# Autodesk Inventor assembly: Final Full Assembly
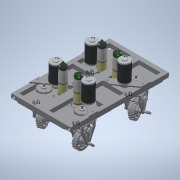
[picture p0: Inventor's stored thumbnail of the model, 180x180]
Saved by Autodesk Inventor 2021 (Build 250183000, 183)
## iProperties
Created: 2018-07-11
Part Number: Final Full Assembly
Document SubType Name: Assembly
Designer: Mortem
Author: Mortem
## Documents named in this file (19)
- C:\Users\PC\Documents\161_VS300_CAD\Final Full Assembly.iam
- F:\GrabCAD\Personal\3D Printed Swerve JP FIRST ATTEMPT\Swerve v4\Test Frame V4.iam
- F:\GrabCAD\Personal\3D Printed Swerve JP FIRST ATTEMPT\Swerve v4\Bottom Plate.ipt
- F:\GrabCAD\Personal\3D Printed Swerve JP FIRST ATTEMPT\Swerve v4\Module Seperate.iam
- F:\GrabCAD\Personal\3D Printed Swerve JP FIRST ATTEMPT\Swerve v4\56t.ipt
- F:\GrabCAD\Personal\3D Printed Swerve JP FIRST ATTEMPT\Swerve v4\cim power spacer.ipt
- F:\GrabCAD\Personal\3D Printed Swerve JP FIRST ATTEMPT\Swerve v4\am-2300+Collar+Clamp,+0.375''+Hex+Bore,+Aluminum.iam
- F:\GrabCAD\Personal\3D Printed Swerve JP FIRST ATTEMPT\Swerve v4\PG71 turning motor.iam
- F:\GrabCAD\Personal\3D Printed Swerve JP FIRST ATTEMPT\Swerve v4\New turning gear.ipt
- F:\GrabCAD\Personal\3D Printed Swerve JP FIRST ATTEMPT\Swerve v4\am-0255+2.5inch+CIM+Motor.ipt
- F:\GrabCAD\Personal\3D Printed Swerve JP FIRST ATTEMPT\Swerve v4\35t.ipt
- F:\GrabCAD\Personal\3D Printed Swerve JP FIRST ATTEMPT\Swerve v4\cim mount.ipt
- F:\GrabCAD\Personal\3D Printed Swerve JP FIRST ATTEMPT\Swerve v4\cim spacer.ipt
- F:\GrabCAD\Personal\3D Printed Swerve JP FIRST ATTEMPT\Swerve v4\motor gear 1-1.ipt
- F:\GrabCAD\Personal\3D Printed Swerve JP FIRST ATTEMPT\Swerve v4\am-0692+FR6ZZL-hex.ipt
- F:\GrabCAD\Personal\3D Printed Swerve JP FIRST ATTEMPT\Swerve v4\Bottom Plate Mirror.ipt
- F:\GrabCAD\Personal\3D Printed Swerve JP FIRST ATTEMPT\Swerve v4\electrical cab.ipt
- F:\GrabCAD\Personal\3D Printed Swerve JP FIRST ATTEMPT\Swerve v4\Talon Holder.ipt
- F:\GrabCAD\Personal\3D Printed Swerve JP FIRST ATTEMPT\Swerve v4\COTS\217-8080-STEP-20140814.ipt
## Components (55 placed, 18 different names)
1. Test Frame V4:1 [sub-assembly] — Mate:1, Flush:1, Flush:2, Mate:13, Mate:14, Mate:20, Flush:5, Flush:6, Mate:32, Flush:7, Mate:53, Flush:8, Flush:9, Mate:58, Flush:10, Flush:11, Mate:59, Flush:12, Flush:13, Mate:67, Flush:14, Mate:68, Flush:15, Flush:16, Mate:114, Mate:115, Flush:17, Mate:116
2. Bottom Plate:1 — Mate:1, Flush:1, Flush:2, Mate:3, Mate:11, Mate:24, Mate:29, Mate:30, Mate:33
3. Module Seperate:1 [sub-assembly] — Mate:3, Flush:3, Mate:15
4. 56t:1 — Mate:8, Mate:10, Mate:16, Mate:17, Flush:4, Rotation:1
5. cim power spacer:1 — Mate:8, Mate:15, Mate:16, Mate:31
6. am-2300+Collar+Clamp,+0.375''+Hex+Bore,+Aluminum:1 [sub-assembly] — Mate:10, Mate:17
7. PG71 turning motor:1 [sub-assembly] — Mate:11, Mate:12, Mate:13, Mate:14, Mate:27, Mate:28
8. New turning gear:1 — Mate:12, Flush:3
9. am-0255+2.5inch+CIM+Motor:1 — Mate:19, Mate:21
10. 35t:1 — Mate:19, Flush:4, Rotation:1, Mate:25, Mate:26
11. cim mount:1 — Mate:20, Flush:5, Flush:6, Mate:21, Mate:26
12. cim spacer:1 — Mate:24, Mate:25
13. motor gear 1-1:1 — Mate:27, Mate:28
14. am-0692+FR6ZZL-hex:1 — Mate:29, Mate:30, Mate:31
15. Bottom Plate Mirror:1 — Mate:32, Flush:7, Mate:33, Mate:34, Mate:35, Mate:36, Mate:41, Mate:42, Mate:43, Mate:44, Mate:45, Mate:52, Mate:117
16. PG71 turning motor:2 [sub-assembly] — Mate:34, Mate:35, Mate:36, Mate:37, Mate:40
17. New turning gear:2 — Mate:38, Mate:39
18. motor gear 1-1:2 — Mate:37, Mate:38, Mate:39, Mate:40
19. Module Seperate:2 [sub-assembly] — Mate:43, Mate:44, Mate:45
20. am-0692+FR6ZZL-hex:2 — Mate:41, Mate:42, Mate:50, Mate:51
21. 56t:2
22. cim power spacer:2 — Mate:50, Mate:51
23. am-2300+Collar+Clamp,+0.375''+Hex+Bore,+Aluminum:2 [sub-assembly]
24. am-0255+2.5inch+CIM+Motor:2 — Mate:52, Mate:54, Mate:56, Mate:57
25. cim mount:2 — Mate:53, Flush:8, Flush:9, Mate:54
26. 35t:2 — Mate:56, Mate:57
27. Bottom Plate:2 — Mate:58, Flush:10, Flush:11, Mate:60, Mate:61, Mate:65, Mate:66, Mate:74, Mate:75, Mate:76, Mate:88, Mate:89, Mate:90, Mate:108
28. Bottom Plate Mirror:2 — Mate:59, Flush:12, Mate:60, Mate:62, Mate:63, Mate:64, Mate:82, Mate:83, Mate:85, Mate:86, Mate:87, Mate:112
29. PG71 turning motor:3 [sub-assembly] — Mate:61, Mate:65, Mate:66, Mate:99, Mate:100, Mate:101, Mate:102
30. PG71 turning motor:4 [sub-assembly] — Mate:62, Mate:63, Mate:64, Mate:95, Mate:96, Mate:97
31. cim mount:3 — Flush:13, Mate:67, Flush:14, Mate:91, Mate:94
32. cim mount:4 — Mate:68, Flush:15, Flush:16, Mate:92, Mate:93, Mate:113
33. 56t:3
34. cim power spacer:3
35. am-2300+Collar+Clamp,+0.375''+Hex+Bore,+Aluminum:3 [sub-assembly] — Mate:74
36. am-0692+FR6ZZL-hex:3 — Mate:75, Mate:76
37. 56t:4
38. cim power spacer:4
39. am-2300+Collar+Clamp,+0.375''+Hex+Bore,+Aluminum:4 [sub-assembly] — Mate:84
40. am-0692+FR6ZZL-hex:4 — Mate:82, Mate:83, Mate:84
41. Module Seperate:3 [sub-assembly] — Mate:88, Mate:89, Mate:90
42. Module Seperate:4 [sub-assembly] — Mate:85, Mate:86, Mate:87
43. am-0255+2.5inch+CIM+Motor:3 — Mate:91, Mate:94, Mate:111
44. am-0255+2.5inch+CIM+Motor:4 — Mate:92, Mate:93, Mate:107
45. New turning gear:3 — Mate:97, Mate:98
46. motor gear 1-1:3 — Mate:95, Mate:96, Mate:98
47. motor gear 1-1:4 — Mate:99, Mate:100, Mate:101, Mate:103
48. New turning gear:4 — Mate:102, Mate:103
49. 35t:3 — Mate:105, Mate:106, Mate:107
50. cim spacer:2 — Mate:105, Mate:106, Mate:108
51. 35t:4 — Mate:110, Mate:111
52. cim spacer:3 — Mate:110, Mate:112
53. electrical cab:1 — Mate:113, Mate:114, Mate:115
54. Talon Holder:1 — Flush:17, Mate:116, Mate:117, Mate:128
55. 217-8080-STEP-20140814:7 — Mate:128
## Relationships (126: Mate 108, Flush 17, RelateRotation 1)
- Mate:1: Test Frame V4:1 ↔ Bottom Plate:1
- Flush:1: Test Frame V4:1 ↔ Bottom Plate:1
- Flush:2: Test Frame V4:1 ↔ Bottom Plate:1
- Mate:3 (16.5862 mm): Bottom Plate:1 ↔ Module Seperate:1
- Mate:8: 56t:1 ↔ cim power spacer:1
- Mate:10: 56t:1 ↔ am-2300+Collar+Clamp,+0.375''+Hex+Bore,+Aluminum:1
- Mate:11: Bottom Plate:1 ↔ PG71 turning motor:1
- Mate:12: PG71 turning motor:1 ↔ New turning gear:1
- Flush:3: Module Seperate:1 ↔ New turning gear:1
- Mate:13: Test Frame V4:1 ↔ PG71 turning motor:1
- Mate:14: Test Frame V4:1 ↔ PG71 turning motor:1
- Mate:15: Module Seperate:1 ↔ cim power spacer:1
- Mate:16: 56t:1 ↔ cim power spacer:1
- Mate:17: 56t:1 ↔ am-2300+Collar+Clamp,+0.375''+Hex+Bore,+Aluminum:1
- Mate:19: am-0255+2.5inch+CIM+Motor:1 ↔ 35t:1
- Flush:4: 56t:1 ↔ 35t:1
- Rotation:1 [RelateRotation] (1.568 ul): 56t:1 ↔ 35t:1
- Mate:20: Test Frame V4:1 ↔ cim mount:1
- Flush:5: Test Frame V4:1 ↔ cim mount:1
- Flush:6: Test Frame V4:1 ↔ cim mount:1
- Mate:21: am-0255+2.5inch+CIM+Motor:1 ↔ cim mount:1
- Mate:24: Bottom Plate:1 ↔ cim spacer:1
- Mate:25: 35t:1 ↔ cim spacer:1
- Mate:26: 35t:1 ↔ cim mount:1
- Mate:27: PG71 turning motor:1 ↔ motor gear 1-1:1
- Mate:28: PG71 turning motor:1 ↔ motor gear 1-1:1
- Mate:29: Bottom Plate:1 ↔ am-0692+FR6ZZL-hex:1
- Mate:30: Bottom Plate:1 ↔ am-0692+FR6ZZL-hex:1
- Mate:31: cim power spacer:1 ↔ am-0692+FR6ZZL-hex:1
- Mate:32: Test Frame V4:1 ↔ Bottom Plate Mirror:1
- Flush:7: Test Frame V4:1 ↔ Bottom Plate Mirror:1
- Mate:33: Bottom Plate:1 ↔ Bottom Plate Mirror:1
- Mate:34: Bottom Plate Mirror:1 ↔ PG71 turning motor:2
- Mate:35: Bottom Plate Mirror:1 ↔ PG71 turning motor:2
- Mate:36: Bottom Plate Mirror:1 ↔ PG71 turning motor:2
- Mate:37: PG71 turning motor:2 ↔ motor gear 1-1:2
- Mate:38: New turning gear:2 ↔ motor gear 1-1:2
- Mate:39: New turning gear:2 ↔ motor gear 1-1:2
- Mate:40: PG71 turning motor:2 ↔ motor gear 1-1:2
- Mate:41: Bottom Plate Mirror:1 ↔ am-0692+FR6ZZL-hex:2
- Mate:42: Bottom Plate Mirror:1 ↔ am-0692+FR6ZZL-hex:2
- Mate:43: Bottom Plate Mirror:1 ↔ Module Seperate:2
- Mate:44: Bottom Plate Mirror:1 ↔ Module Seperate:2
- Mate:45: Bottom Plate Mirror:1 ↔ Module Seperate:2
- [Mate]: 56t:2 ↔ cim power spacer:2
- [Mate]: 56t:2 ↔ am-2300+Collar+Clamp,+0.375''+Hex+Bore,+Aluminum:2
- [Mate]: 56t:2 ↔ cim power spacer:2
- [Mate]: 56t:2 ↔ am-2300+Collar+Clamp,+0.375''+Hex+Bore,+Aluminum:2
- Mate:50: am-0692+FR6ZZL-hex:2 ↔ cim power spacer:2
- Mate:51: am-0692+FR6ZZL-hex:2 ↔ cim power spacer:2
- Mate:52: Bottom Plate Mirror:1 ↔ am-0255+2.5inch+CIM+Motor:2
- Mate:53: Test Frame V4:1 ↔ cim mount:2
- Flush:8: Test Frame V4:1 ↔ cim mount:2
- Flush:9: Test Frame V4:1 ↔ cim mount:2
- Mate:54: am-0255+2.5inch+CIM+Motor:2 ↔ cim mount:2
- Mate:56: am-0255+2.5inch+CIM+Motor:2 ↔ 35t:2
- Mate:57: am-0255+2.5inch+CIM+Motor:2 ↔ 35t:2
- Mate:58: Test Frame V4:1 ↔ Bottom Plate:2
- Flush:10: Test Frame V4:1 ↔ Bottom Plate:2
- Flush:11: Test Frame V4:1 ↔ Bottom Plate:2
- Mate:59: Test Frame V4:1 ↔ Bottom Plate Mirror:2
- Flush:12: Test Frame V4:1 ↔ Bottom Plate Mirror:2
- Mate:60: Bottom Plate:2 ↔ Bottom Plate Mirror:2
- Mate:61: Bottom Plate:2 ↔ PG71 turning motor:3
- Mate:62: Bottom Plate Mirror:2 ↔ PG71 turning motor:4
- Mate:63: Bottom Plate Mirror:2 ↔ PG71 turning motor:4
- Mate:64: Bottom Plate Mirror:2 ↔ PG71 turning motor:4
- Mate:65: Bottom Plate:2 ↔ PG71 turning motor:3
- Mate:66: Bottom Plate:2 ↔ PG71 turning motor:3
- Flush:13: Test Frame V4:1 ↔ cim mount:3
- Mate:67: Test Frame V4:1 ↔ cim mount:3
- Flush:14: Test Frame V4:1 ↔ cim mount:3
- Mate:68: Test Frame V4:1 ↔ cim mount:4
- Flush:15: Test Frame V4:1 ↔ cim mount:4
- Flush:16: Test Frame V4:1 ↔ cim mount:4
- [Mate]: 56t:3 ↔ cim power spacer:3
- [Mate]: 56t:3 ↔ am-2300+Collar+Clamp,+0.375''+Hex+Bore,+Aluminum:3
- [Mate]: 56t:3 ↔ cim power spacer:3
- [Mate]: 56t:3 ↔ am-2300+Collar+Clamp,+0.375''+Hex+Bore,+Aluminum:3
- [Mate]: cim power spacer:3 ↔ am-0692+FR6ZZL-hex:3
- Mate:74: Bottom Plate:2 ↔ am-2300+Collar+Clamp,+0.375''+Hex+Bore,+Aluminum:3
- Mate:75: Bottom Plate:2 ↔ am-0692+FR6ZZL-hex:3
- Mate:76: Bottom Plate:2 ↔ am-0692+FR6ZZL-hex:3
- [Mate]: 56t:4 ↔ cim power spacer:4
- [Mate]: 56t:4 ↔ am-2300+Collar+Clamp,+0.375''+Hex+Bore,+Aluminum:4
- [Mate]: 56t:4 ↔ cim power spacer:4
- [Mate]: 56t:4 ↔ am-2300+Collar+Clamp,+0.375''+Hex+Bore,+Aluminum:4
- [Mate]: cim power spacer:4 ↔ am-0692+FR6ZZL-hex:4
- Mate:82: Bottom Plate Mirror:2 ↔ am-0692+FR6ZZL-hex:4
- Mate:83: Bottom Plate Mirror:2 ↔ am-0692+FR6ZZL-hex:4
- Mate:84: am-2300+Collar+Clamp,+0.375''+Hex+Bore,+Aluminum:4 ↔ am-0692+FR6ZZL-hex:4
- Mate:85: Bottom Plate Mirror:2 ↔ Module Seperate:4
- Mate:86: Bottom Plate Mirror:2 ↔ Module Seperate:4
- Mate:87: Bottom Plate Mirror:2 ↔ Module Seperate:4
- Mate:88: Bottom Plate:2 ↔ Module Seperate:3
- Mate:89: Bottom Plate:2 ↔ Module Seperate:3
- Mate:90: Bottom Plate:2 ↔ Module Seperate:3
- Mate:91: cim mount:3 ↔ am-0255+2.5inch+CIM+Motor:3
- Mate:92: cim mount:4 ↔ am-0255+2.5inch+CIM+Motor:4
- Mate:93: cim mount:4 ↔ am-0255+2.5inch+CIM+Motor:4
- Mate:94: cim mount:3 ↔ am-0255+2.5inch+CIM+Motor:3
- Mate:95: PG71 turning motor:4 ↔ motor gear 1-1:3
- Mate:96: PG71 turning motor:4 ↔ motor gear 1-1:3
- Mate:97: PG71 turning motor:4 ↔ New turning gear:3
- Mate:98: New turning gear:3 ↔ motor gear 1-1:3
- Mate:99: PG71 turning motor:3 ↔ motor gear 1-1:4
- Mate:100: PG71 turning motor:3 ↔ motor gear 1-1:4
- Mate:101: PG71 turning motor:3 ↔ motor gear 1-1:4
- Mate:102: PG71 turning motor:3 ↔ New turning gear:4
- Mate:103: motor gear 1-1:4 ↔ New turning gear:4
- [Mate]: 35t:3 ↔ cim spacer:2
- Mate:105: 35t:3 ↔ cim spacer:2
- Mate:106: 35t:3 ↔ cim spacer:2
- Mate:107: am-0255+2.5inch+CIM+Motor:4 ↔ 35t:3
- Mate:108: Bottom Plate:2 ↔ cim spacer:2
- [Mate]: 35t:4 ↔ cim spacer:3
- Mate:110: 35t:4 ↔ cim spacer:3
- Mate:111: am-0255+2.5inch+CIM+Motor:3 ↔ 35t:4
- Mate:112: Bottom Plate Mirror:2 ↔ cim spacer:3
- Mate:113: cim mount:4 ↔ electrical cab:1
- Mate:114 (-304.8 mm): Test Frame V4:1 ↔ electrical cab:1
- Mate:115 (-184.15 mm): Test Frame V4:1 ↔ electrical cab:1
- Flush:17: Test Frame V4:1 ↔ Talon Holder:1
- Mate:116: Test Frame V4:1 ↔ Talon Holder:1
- Mate:117: Bottom Plate Mirror:1 ↔ Talon Holder:1
- Mate:128: Talon Holder:1 ↔ 217-8080-STEP-20140814:7
## Named parameters: d56_d10 = 0 mm, d57_d12 = 0 mm, d58_d19 = 0 mm, d59_d20 = 0 mm, d89_d40 = 0 mm, d90_d10 = 0 mm, d91_d12 = 0 mm, d92_d19 = 0 mm, d93_d20 = 0 mm, d97_d40 = 0 mm, d98_d10 = 0 mm, d99_d12 = 0 mm, d100_d19 = 0 mm, d101_d20 = 0 mm, d124_d34 = 0 mm, d129_d34 = 0 mm
